# Autodesk Inventor assembly: Zespół1
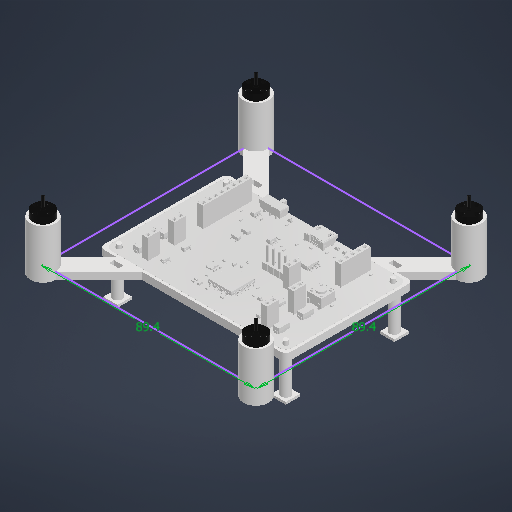
[picture p0: Inventor's stored thumbnail of the model, 512x512]
Saved by Autodesk Inventor 2026 (Build 300175050, 175E)
## iProperties
Created: 2026-01-10
Part Number: Zespół1
Document SubType Name: Assembly
Designer: DeathLock
Author: DeathLock
## Documents named in this file (4)
- E:\DeathProject\Praca Inżynierska\STM32-Drone\Drone_3D\Zespół1.iam
- E:\DeathProject\Praca Inżynierska\STM32-Drone\Drone_3D\8520 Coreless Brshed motor.ipt
- E:\DeathProject\Praca Inżynierska\STM32-Drone\Drone_3D\Drone.ipt
- E:\DeathProject\Praca Inżynierska\STM32-Drone\Drone_3D\Drone_PCB.ipt
## Components (6 placed, 3 different names)
1. Drone:1 — Sztywne:1, Sztywne:4, Sztywne:5, Sztywne:6, Sztywne:7, Sztywne:10, Sztywne:13, Sztywne:14, Sztywne:15
2. Drone_PCB:1 — Sztywne:1, Sztywne:6
3. 8520 Coreless Brshed motor:1
4. 8520 Coreless Brshed motor:2 — Sztywne:4, Sztywne:7, Sztywne:13
5. 8520 Coreless Brshed motor:3 — Sztywne:5, Sztywne:10, Sztywne:14
6. 8520 Coreless Brshed motor:4 — Sztywne:15
## Relationships (9: WeldJoint 9)
- Sztywne:1 [WeldJoint]: Drone:1 ↔ Drone_PCB:1
- Sztywne:4 [WeldJoint]: Drone:1 ↔ 8520 Coreless Brshed motor:2
- Sztywne:5 [WeldJoint]: Drone:1 ↔ 8520 Coreless Brshed motor:3
- Sztywne:6 [WeldJoint]: Drone:1 ↔ Drone_PCB:1
- Sztywne:7 [WeldJoint]: Drone:1 ↔ 8520 Coreless Brshed motor:2
- Sztywne:10 [WeldJoint]: Drone:1 ↔ 8520 Coreless Brshed motor:3
- Sztywne:13 [WeldJoint]: Drone:1 ↔ 8520 Coreless Brshed motor:2
- Sztywne:14 [WeldJoint]: Drone:1 ↔ 8520 Coreless Brshed motor:3
- Sztywne:15 [WeldJoint]: Drone:1 ↔ 8520 Coreless Brshed motor:4
